# Autodesk Inventor assembly: StackAvionics_V2
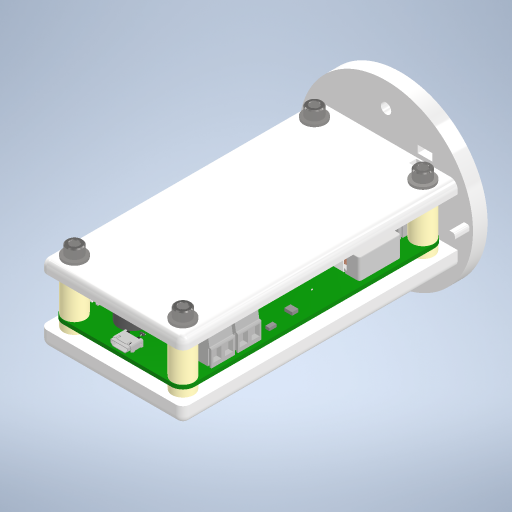
[picture p0: Inventor's stored thumbnail of the model, 512x512]
Saved by Autodesk Inventor 2023 (Build 270158000, 158)
## iProperties
Created: 2022-10-05
Part Number: StackAvionics_V2
Document SubType Name: Assembly
Designer: jeanp
Author: jeanp
## Documents named in this file (10)
- C:\Users\jeanp\Documents\ETS\RockETS\Certification JEEP\Avionics\StackAvionics_V2.iam
- C:\Users\jeanp\Documents\ETS\RockETS\Certification JEEP\Avionics\Supportv2_3dprinted.ipt
- C:\Users\jeanp\Documents\ETS\RockETS\Certification JEEP\Avionics\92395A324_Brass Screw-to-Expand Inserts.ipt
- C:\Users\jeanp\Documents\ETS\RockETS\Certification JEEP\Avionics\mini-rocket.ipt
- C:\Users\jeanp\Documents\ETS\RockETS\Certification JEEP\Avionics\94639A427_Off-White Nylon Unthreaded Spacer.ipt
- C:\Users\jeanp\Documents\ETS\RockETS\Certification JEEP\Avionics\94639A404_Off-White Nylon Unthreaded Spacer.ipt
- C:\Users\jeanp\Documents\ETS\RockETS\Certification JEEP\Avionics\92141A009_18-8 Stainless Steel Washer.ipt
- C:\Users\jeanp\Documents\ETS\RockETS\Certification JEEP\Avionics\91864A026_Black-Oxide Alloy Steel Socket Head Screw.ipt
- C:\Users\jeanp\Documents\ETS\RockETS\Certification JEEP\Avionics\9V-battery.ipt
- C:\Users\jeanp\Documents\ETS\RockETS\Certification JEEP\Avionics\BatteryHolder_DigiKEY.ipt
## Components (24 placed, 9 different names)
1. Supportv2_3dprinted:1 — Mate:1, Mate:2, Mate:3, Mate:4, Mate:5, Mate:6, Mate:7, Mate:8, Angle:1, Mate:11, Mate:12, Mate:14, Mate:16, Mate:17, Mate:27, Mate:28, Mate:29, Mate:30, Mate:31, Mate:32, Mate:33, Mate:34, Mate:46, Flush:1
2. 92395A324_Brass Screw-to-Expand Inserts:1 — Mate:1, Mate:2, Mate:9, Mate:10
3. 92395A324_Brass Screw-to-Expand Inserts:2 — Mate:3, Mate:4, Mate:13
4. 92395A324_Brass Screw-to-Expand Inserts:3 — Mate:5, Mate:6
5. 92395A324_Brass Screw-to-Expand Inserts:4 — Mate:7, Mate:8, Mate:15
6. mini-rocket:1 — Mate:9, Angle:1, Mate:18, Mate:19, Mate:20, Mate:21, Mate:22, Mate:23, Mate:24, Mate:25, Mate:26
7. 94639A427_Off-White Nylon Unthreaded Spacer:1 — Mate:10, Mate:11, Mate:18
8. 94639A427_Off-White Nylon Unthreaded Spacer:2 — Mate:12, Mate:13
9. 94639A427_Off-White Nylon Unthreaded Spacer:3 — Mate:14, Mate:15
10. 94639A427_Off-White Nylon Unthreaded Spacer:4 — Mate:16, Mate:17
11. 94639A404_Off-White Nylon Unthreaded Spacer:1 — Mate:19, Mate:20
12. 94639A404_Off-White Nylon Unthreaded Spacer:2 — Mate:21, Mate:22
13. 94639A404_Off-White Nylon Unthreaded Spacer:3 — Mate:23, Mate:24
14. 94639A404_Off-White Nylon Unthreaded Spacer:4 — Mate:25, Mate:26
15. 92141A009_18-8 Stainless Steel Washer:1 — Mate:27, Mate:28, Mate:35, Mate:36
16. 92141A009_18-8 Stainless Steel Washer:2 — Mate:29, Mate:30, Mate:37, Mate:38
17. 92141A009_18-8 Stainless Steel Washer:3 — Mate:33, Mate:34, Mate:39, Mate:40
18. 92141A009_18-8 Stainless Steel Washer:4 — Mate:31, Mate:32, Mate:41, Mate:42
19. 91864A026_Black-Oxide Alloy Steel Socket Head Screw:1 — Mate:35, Mate:36
20. 91864A026_Black-Oxide Alloy Steel Socket Head Screw:2 — Mate:37, Mate:38
21. 91864A026_Black-Oxide Alloy Steel Socket Head Screw:3 — Mate:41, Mate:42
22. 91864A026_Black-Oxide Alloy Steel Socket Head Screw:4 — Mate:39, Mate:40
23. 9V-battery:1 — Mate:47, Mate:48
24. BatteryHolder_DigiKEY:1 — Mate:46, Angle:4, Flush:1, Mate:47, Mate:48
## Relationships (48: Mate 45, Angle 2, Flush 1)
- Mate:1: Supportv2_3dprinted:1 ↔ 92395A324_Brass Screw-to-Expand Inserts:1
- Mate:2: Supportv2_3dprinted:1 ↔ 92395A324_Brass Screw-to-Expand Inserts:1
- Mate:3: Supportv2_3dprinted:1 ↔ 92395A324_Brass Screw-to-Expand Inserts:2
- Mate:4: Supportv2_3dprinted:1 ↔ 92395A324_Brass Screw-to-Expand Inserts:2
- Mate:5: Supportv2_3dprinted:1 ↔ 92395A324_Brass Screw-to-Expand Inserts:3
- Mate:6: Supportv2_3dprinted:1 ↔ 92395A324_Brass Screw-to-Expand Inserts:3
- Mate:7: Supportv2_3dprinted:1 ↔ 92395A324_Brass Screw-to-Expand Inserts:4
- Mate:8: Supportv2_3dprinted:1 ↔ 92395A324_Brass Screw-to-Expand Inserts:4
- Mate:9: 92395A324_Brass Screw-to-Expand Inserts:1 ↔ mini-rocket:1
- Angle:1 (0 deg): Supportv2_3dprinted:1 ↔ mini-rocket:1
- Mate:10: 92395A324_Brass Screw-to-Expand Inserts:1 ↔ 94639A427_Off-White Nylon Unthreaded Spacer:1
- Mate:11: Supportv2_3dprinted:1 ↔ 94639A427_Off-White Nylon Unthreaded Spacer:1
- Mate:12: Supportv2_3dprinted:1 ↔ 94639A427_Off-White Nylon Unthreaded Spacer:2
- Mate:13: 92395A324_Brass Screw-to-Expand Inserts:2 ↔ 94639A427_Off-White Nylon Unthreaded Spacer:2
- Mate:14: Supportv2_3dprinted:1 ↔ 94639A427_Off-White Nylon Unthreaded Spacer:3
- Mate:15: 92395A324_Brass Screw-to-Expand Inserts:4 ↔ 94639A427_Off-White Nylon Unthreaded Spacer:3
- Mate:16: Supportv2_3dprinted:1 ↔ 94639A427_Off-White Nylon Unthreaded Spacer:4
- Mate:17: Supportv2_3dprinted:1 ↔ 94639A427_Off-White Nylon Unthreaded Spacer:4
- Mate:18: mini-rocket:1 ↔ 94639A427_Off-White Nylon Unthreaded Spacer:1
- Mate:19: mini-rocket:1 ↔ 94639A404_Off-White Nylon Unthreaded Spacer:1
- Mate:20: mini-rocket:1 ↔ 94639A404_Off-White Nylon Unthreaded Spacer:1
- Mate:21: mini-rocket:1 ↔ 94639A404_Off-White Nylon Unthreaded Spacer:2
- Mate:22: mini-rocket:1 ↔ 94639A404_Off-White Nylon Unthreaded Spacer:2
- Mate:23: mini-rocket:1 ↔ 94639A404_Off-White Nylon Unthreaded Spacer:3
- Mate:24: mini-rocket:1 ↔ 94639A404_Off-White Nylon Unthreaded Spacer:3
- Mate:25: mini-rocket:1 ↔ 94639A404_Off-White Nylon Unthreaded Spacer:4
- Mate:26: mini-rocket:1 ↔ 94639A404_Off-White Nylon Unthreaded Spacer:4
- Mate:27: Supportv2_3dprinted:1 ↔ 92141A009_18-8 Stainless Steel Washer:1
- Mate:28: Supportv2_3dprinted:1 ↔ 92141A009_18-8 Stainless Steel Washer:1
- Mate:29: Supportv2_3dprinted:1 ↔ 92141A009_18-8 Stainless Steel Washer:2
- Mate:30: Supportv2_3dprinted:1 ↔ 92141A009_18-8 Stainless Steel Washer:2
- Mate:31: Supportv2_3dprinted:1 ↔ 92141A009_18-8 Stainless Steel Washer:4
- Mate:32: Supportv2_3dprinted:1 ↔ 92141A009_18-8 Stainless Steel Washer:4
- Mate:33: Supportv2_3dprinted:1 ↔ 92141A009_18-8 Stainless Steel Washer:3
- Mate:34: Supportv2_3dprinted:1 ↔ 92141A009_18-8 Stainless Steel Washer:3
- Mate:35: 92141A009_18-8 Stainless Steel Washer:1 ↔ 91864A026_Black-Oxide Alloy Steel Socket Head Screw:1
- Mate:36: 92141A009_18-8 Stainless Steel Washer:1 ↔ 91864A026_Black-Oxide Alloy Steel Socket Head Screw:1
- Mate:37: 92141A009_18-8 Stainless Steel Washer:2 ↔ 91864A026_Black-Oxide Alloy Steel Socket Head Screw:2
- Mate:38: 92141A009_18-8 Stainless Steel Washer:2 ↔ 91864A026_Black-Oxide Alloy Steel Socket Head Screw:2
- Mate:39: 92141A009_18-8 Stainless Steel Washer:3 ↔ 91864A026_Black-Oxide Alloy Steel Socket Head Screw:4
- Mate:40: 92141A009_18-8 Stainless Steel Washer:3 ↔ 91864A026_Black-Oxide Alloy Steel Socket Head Screw:4
- Mate:41: 92141A009_18-8 Stainless Steel Washer:4 ↔ 91864A026_Black-Oxide Alloy Steel Socket Head Screw:3
- Mate:42: 92141A009_18-8 Stainless Steel Washer:4 ↔ 91864A026_Black-Oxide Alloy Steel Socket Head Screw:3
- Mate:46: Supportv2_3dprinted:1 ↔ BatteryHolder_DigiKEY:1
- Angle:4 (0 deg): BatteryHolder_DigiKEY:1
- Flush:1: Supportv2_3dprinted:1 ↔ BatteryHolder_DigiKEY:1
- Mate:47 (2.54 mm): 9V-battery:1 ↔ BatteryHolder_DigiKEY:1
- Mate:48 (2.54 mm): 9V-battery:1 ↔ BatteryHolder_DigiKEY:1
